# Autodesk Inventor assembly: Top Assembly
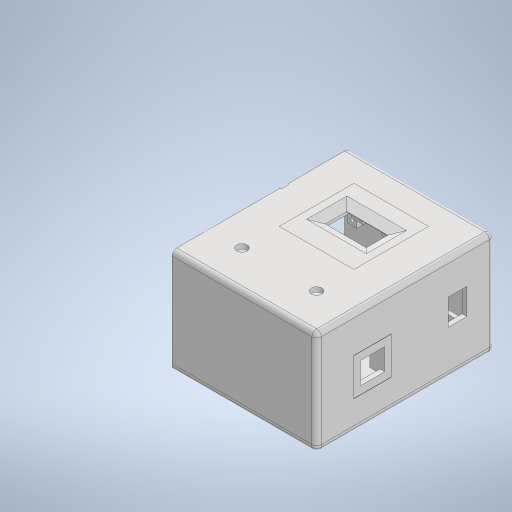
[picture p0: Inventor's stored thumbnail of the model, 512x512]
Saved by Autodesk Inventor 2024 (Build 280153000, 153)
## iProperties
Created: 2025-09-23
Part Number: Top Assembly
Document SubType Name: Assembly
Designer: Martin
Author: Martin
## Documents named in this file (6)
- D:\Users\Martin\OneDrive\Work\Inventor\W2Lab\StageDriver\Top Assembly.iam
- D:\Users\Martin\OneDrive\Work\Inventor\W2Lab\StageDriver\RemoteControllerTop.ipt
- D:\Users\Martin\OneDrive\Work\Inventor\W2Lab\StageDriver\DisplayInsert.ipt
- D:\Users\Martin\OneDrive\Work\Inventor\W2Lab\StageDriver\JoystickInsert.ipt
- D:\Users\Martin\OneDrive\Work\Inventor\W2Lab\StageDriver\RJ45Insert.ipt
- D:\Users\Martin\OneDrive\Work\Inventor\W2Lab\StageDriver\RemoteControllerBottom.ipt
## Components (5 placed, 5 different names)
1. RemoteControllerTop:1 — Mate:1, Mate:2, Flush:1, Mate:3, Flush:2, Mate:5, Mate:6, Flush:3, Mate:7, Mate:8, Flush:4, Flush:5
2. DisplayInsert:1 — Mate:3, Flush:2, Mate:7
3. RJ45Insert:1 — Mate:1, Mate:2, Flush:1
4. JoystickInsert:1 — Mate:5, Mate:6, Flush:3
5. RemoteControllerBottom:1 — Mate:8, Flush:4, Flush:5
## Relationships (12: Mate 7, Flush 5)
- Mate:1: RemoteControllerTop:1 ↔ RJ45Insert:1
- Mate:2: RemoteControllerTop:1 ↔ RJ45Insert:1
- Flush:1: RemoteControllerTop:1 ↔ RJ45Insert:1
- Mate:3: RemoteControllerTop:1 ↔ DisplayInsert:1
- Flush:2: RemoteControllerTop:1 ↔ DisplayInsert:1
- Mate:5: RemoteControllerTop:1 ↔ JoystickInsert:1
- Mate:6: RemoteControllerTop:1 ↔ JoystickInsert:1
- Flush:3: RemoteControllerTop:1 ↔ JoystickInsert:1
- Mate:7: RemoteControllerTop:1 ↔ DisplayInsert:1
- Mate:8: RemoteControllerTop:1 ↔ RemoteControllerBottom:1
- Flush:4: RemoteControllerTop:1 ↔ RemoteControllerBottom:1
- Flush:5: RemoteControllerTop:1 ↔ RemoteControllerBottom:1
